# Autodesk Inventor assembly: Этаж 1
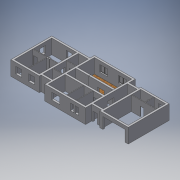
[picture p0: Inventor's stored thumbnail of the model, 180x180]
Saved by Autodesk Inventor 2019 (Build 230136000, 136)
## iProperties
Created: 2018-09-18
Part Number: Этаж 1
Material: Типовые
Document SubType Name: Assembly
Designer: Андреев Н.Л.
Author: Андреев Н.Л.
## Documents named in this file (6)
- C:\Users\andrnl\Documents\Inventor\Мурзин\Этаж 1.iam
- C:\Users\andrnl\Documents\Inventor\Мурзин\Этаж 1.ipt
- C:\Users\andrnl\Documents\Inventor\Мурзин\Окно 2 рамы\Окно 2 рамы-01.ipt
- C:\Users\andrnl\Documents\Inventor\Мурзин\Окно 2 рамы.ipt
- C:\Users\andrnl\Documents\Inventor\Мурзин\Пол гостиной.ipt
- C:\Users\andrnl\Documents\Inventor\Мурзин\Перекрытие гостиной.ipt
## Components (5 placed, 4 different names)
1. Этаж 1:1 — Совмещение:1, Совмещение:2, Заподлицо:1, Заподлицо:3
2. Пол гостиной:1 — Заподлицо:2
3. Перекрытие гостиной:1 — Заподлицо:3
4. Окно 2 рамы-01:1 — Совмещение:1, Совмещение:2, Заподлицо:1
5. Окно 2 рамы-01:2
## Component patterns: Окна гостиной:1 (2 elements)
## Relationships (5: Flush 3, Mate 2)
- Совмещение:1 [Mate]: Этаж 1:1 ↔ Окно 2 рамы-01:1
- Совмещение:2 [Mate]: Этаж 1:1 ↔ Окно 2 рамы-01:1
- Заподлицо:1 [Flush] (100 mm): Этаж 1:1 ↔ Окно 2 рамы-01:1
- Заподлицо:2 [Flush]: Пол гостиной:1
- Заподлицо:3 [Flush]: Этаж 1:1 ↔ Перекрытие гостиной:1
